# Autodesk Inventor assembly: Chest Assembly
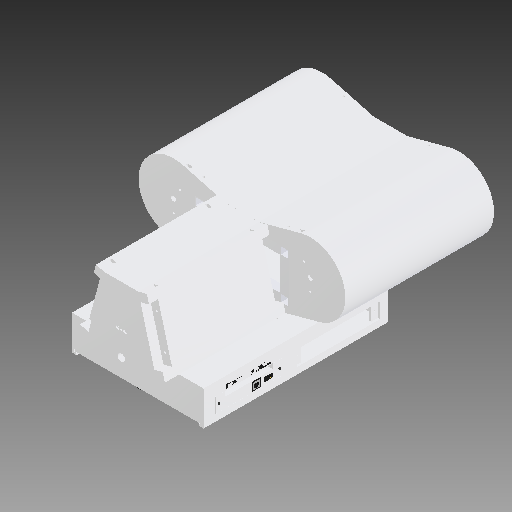
[picture p0: Inventor's stored thumbnail of the model, 512x512]
Saved by Autodesk Inventor 2017 SP1 (Build 210196100, 196)
## iProperties
Created: 2017-06-04
Part Number: Chest Assembly
Document SubType Name: Assembly
Designer: Zach
Author: Zach
## Documents named in this file (5)
- C:\Users\Zach\Documents\GitHub\tr1\src\Body\Chest Assembly\Chest Assembly.iam
- C:\Users\Zach\Documents\GitHub\tr1\src\Body\Chest Assembly\Chassis\Chassis.iam
- C:\Users\Zach\Documents\GitHub\tr1\src\Body\Chest Assembly\Backpack Assembly\Backpack.iam
- C:\Users\Zach\Documents\GitHub\tr1\src\Body\Chest Assembly\Sternum Assembly\Sternum Assembly.iam
- C:\Users\Zach\Documents\GitHub\tr1\src\Body\Chest Assembly\Torso - Solid\Torso Solid.iam
## Components (4 placed, 4 different names)
1. Chassis:1 [sub-assembly] — Flush:1, Mate:32, Mate:33
2. Backpack:1 [sub-assembly] — Mate:36, Mate:37, Mate:38
3. Sternum Assembly:1 [sub-assembly] — Mate:34, Mate:35, Mate:36, Mate:37, Mate:38
4. Torso Solid:1 [sub-assembly] — Flush:1, Mate:32, Mate:33, Mate:34, Mate:35
## Relationships (8: Mate 7, Flush 1)
- Flush:1: Chassis:1 ↔ Torso Solid:1
- Mate:32: Chassis:1 ↔ Torso Solid:1
- Mate:33: Chassis:1 ↔ Torso Solid:1
- Mate:34: Sternum Assembly:1 ↔ Torso Solid:1
- Mate:35: Sternum Assembly:1 ↔ Torso Solid:1
- Mate:36: Backpack:1 ↔ Sternum Assembly:1
- Mate:37: Backpack:1 ↔ Sternum Assembly:1
- Mate:38: Backpack:1 ↔ Sternum Assembly:1
